# Autodesk Inventor assembly: montaje carro  extrusor
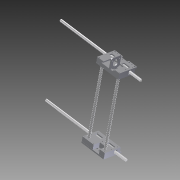
[picture p0: Inventor's stored thumbnail of the model, 180x180]
Saved by Autodesk Inventor 2012 (Build 160160000, 160)
## iProperties
Created: 2014-12-17
Part Number: montaje carro  extrusor
Document SubType Name: Assembly
Designer: PRINCIPAL
Author: PRINCIPAL
## Documents named in this file (16)
- \\LASERROUTERCNC\Users\Laser router cnc\Desktop\compartir con principal\impresora juan marc albert\montaje carro  extrusor.iam
- \\LASERROUTERCNC\Users\Laser router cnc\Desktop\compartir con principal\impresora juan marc albert\carro x lado polea pieza1.ipt
- \\LASERROUTERCNC\Users\Laser router cnc\Desktop\compartir con principal\impresora juan marc albert\carro x lado polea pieza2.ipt
- \\LASERROUTERCNC\Users\Laser router cnc\Desktop\compartir con principal\impresora juan marc albert\carro x lado polea pieza3.ipt
- \\LASERROUTERCNC\Users\Laser router cnc\Desktop\compartir con principal\impresora juan marc albert\carro x lado polea pieza4 tapa.ipt
- \\LASERROUTERCNC\Users\Laser router cnc\Desktop\compartir con principal\impresora juan marc albert\cojinete lm10uu.ipt
- \\LASERROUTERCNC\Users\Laser router cnc\Desktop\compartir con principal\impresora juan marc albert\carro x lado motor pieza 1.ipt
- \\LASERROUTERCNC\Users\Laser router cnc\Desktop\compartir con principal\impresora juan marc albert\carro x lado motor pieza 2 especial2.ipt
- \\LASERROUTERCNC\Users\Laser router cnc\Desktop\compartir con principal\impresora juan marc albert\carro x lado motor pieza 2parte 2.ipt
- \\LASERROUTERCNC\Users\Laser router cnc\Desktop\compartir con principal\impresora juan marc albert\carro x lado motor pieza 2parte 2-2.ipt
- \\LASERROUTERCNC\Users\Laser router cnc\Desktop\compartir con principal\impresora juan marc albert\carro x lado motor pieza 2parte 2-3.ipt
- \\LASERROUTERCNC\Users\Laser router cnc\Desktop\compartir con principal\impresora juan marc albert\carro x lado motor pieza 3.ipt
- \\LASERROUTERCNC\Users\Laser router cnc\Desktop\compartir con principal\impresora juan marc albert\carro x lado motor pieza 4.ipt
- \\LASERROUTERCNC\Users\Laser router cnc\Desktop\compartir con principal\impresora juan marc albert\carro x lado motor pieza 5 soporte nema.ipt
- \\LASERROUTERCNC\Users\Laser router cnc\Desktop\compartir con principal\impresora juan marc albert\varilla 10 carro x.ipt
- \\LASERROUTERCNC\Users\Laser router cnc\Desktop\compartir con principal\impresora juan marc albert\varilla 10 carro y.ipt
## Components (28 placed, 15 different names)
1. carro x lado polea pieza1:1 — Coincidencia:1, Coincidencia:2, Tangente:1, Tangente:2, Tangente:3, Tangente:4, Insertar:1, Insertar:2, Insertar:7, Insertar:8
2. carro x lado polea pieza2:1 — Insertar:7, Insertar:8, Insertar:9, Insertar:10, Insertar:45, Insertar:46
3. carro x lado polea pieza2:2 — Insertar:11, Insertar:12, Insertar:14
4. carro x lado polea pieza2:3 — Insertar:9, Insertar:10, Insertar:11, Insertar:12
5. carro x lado polea pieza3:1 — Insertar:5, Insertar:6, Insertar:13
6. carro x lado polea pieza3:2 — Insertar:3, Insertar:4, Insertar:5, Insertar:6
7. carro x lado polea pieza3:3 — Insertar:1, Insertar:2, Insertar:3, Insertar:4
8. carro x lado polea pieza4 tapa:1 — Insertar:13, Insertar:14
9. cojinete lm10uu:1 — Coincidencia:1, Tangente:3, Tangente:4
10. cojinete lm10uu:2 — Coincidencia:2, Tangente:1, Tangente:2, Insertar:48
11. carro x lado motor pieza 1:1 — Coincidencia:3, Coincidencia:4, Tangente:5, Tangente:6, Tangente:7, Tangente:8, Insertar:17, Insertar:18, Insertar:31, Insertar:32, Insertar:33, Insertar:34
12. carro x lado motor pieza 2 especial2:2 — Insertar:33, Insertar:34, Insertar:35, Insertar:36, Insertar:44
13. carro x lado motor pieza 2parte 2:1 — Insertar:29, Insertar:30, Insertar:41
14. carro x lado motor pieza 2parte 2:2 — Insertar:29, Insertar:30, Insertar:37, Insertar:38
15. carro x lado motor pieza 2parte 2-2:1 — Insertar:25, Insertar:26, Insertar:40
16. carro x lado motor pieza 2parte 2-2:2 — Insertar:25, Insertar:26, Insertar:35, Insertar:36
17. carro x lado motor pieza 2parte 2-3:1 — Insertar:31, Insertar:32, Insertar:37, Insertar:38, Insertar:42
18. carro x lado motor pieza 3:1 — Insertar:17, Insertar:18, Insertar:19, Insertar:20
19. carro x lado motor pieza 3:2 — Insertar:21, Insertar:22, Insertar:39
20. carro x lado motor pieza 3:3 — Insertar:19, Insertar:20, Insertar:21, Insertar:22
21. carro x lado motor pieza 4:1 — Insertar:39, Insertar:40, Insertar:41, Nivelación:1, Coincidencia:5, Coincidencia:6
22. carro x lado motor pieza 5 soporte nema:1 — Nivelación:1, Coincidencia:5, Coincidencia:6
23. cojinete lm10uu:3 — Coincidencia:4, Tangente:7, Tangente:8
24. cojinete lm10uu:4 — Coincidencia:3, Tangente:5, Tangente:6, Insertar:47
25. varilla 10 carro x:1 — Insertar:42, Insertar:46
26. varilla 10 carro x:2 — Insertar:44, Insertar:45
27. varilla 10 carro y:1 — Insertar:47
28. varilla 10 carro y:2 — Insertar:48
## Relationships (56: Insert 41, Tangent 8, Mate 6, Flush 1)
- Coincidencia:1 [Mate]: carro x lado polea pieza1:1 ↔ cojinete lm10uu:1
- Coincidencia:2 [Mate]: carro x lado polea pieza1:1 ↔ cojinete lm10uu:2
- Tangente:1: carro x lado polea pieza1:1 ↔ cojinete lm10uu:2
- Tangente:2: carro x lado polea pieza1:1 ↔ cojinete lm10uu:2
- Tangente:3: carro x lado polea pieza1:1 ↔ cojinete lm10uu:1
- Tangente:4: carro x lado polea pieza1:1 ↔ cojinete lm10uu:1
- Insertar:1: carro x lado polea pieza1:1 ↔ carro x lado polea pieza3:3
- Insertar:2: carro x lado polea pieza1:1 ↔ carro x lado polea pieza3:3
- Insertar:3: carro x lado polea pieza3:2 ↔ carro x lado polea pieza3:3
- Insertar:4: carro x lado polea pieza3:2 ↔ carro x lado polea pieza3:3
- Insertar:5: carro x lado polea pieza3:1 ↔ carro x lado polea pieza3:2
- Insertar:6: carro x lado polea pieza3:1 ↔ carro x lado polea pieza3:2
- Insertar:7: carro x lado polea pieza1:1 ↔ carro x lado polea pieza2:1
- Insertar:8: carro x lado polea pieza1:1 ↔ carro x lado polea pieza2:1
- Insertar:9: carro x lado polea pieza2:1 ↔ carro x lado polea pieza2:3
- Insertar:10: carro x lado polea pieza2:1 ↔ carro x lado polea pieza2:3
- Insertar:11: carro x lado polea pieza2:2 ↔ carro x lado polea pieza2:3
- Insertar:12: carro x lado polea pieza2:2 ↔ carro x lado polea pieza2:3
- Insertar:13: carro x lado polea pieza3:1 ↔ carro x lado polea pieza4 tapa:1
- Insertar:14: carro x lado polea pieza2:2 ↔ carro x lado polea pieza4 tapa:1
- Coincidencia:3 [Mate]: carro x lado motor pieza 1:1 ↔ cojinete lm10uu:4
- Coincidencia:4 [Mate]: carro x lado motor pieza 1:1 ↔ cojinete lm10uu:3
- Tangente:5: carro x lado motor pieza 1:1 ↔ cojinete lm10uu:4
- Tangente:6: carro x lado motor pieza 1:1 ↔ cojinete lm10uu:4
- Tangente:7: carro x lado motor pieza 1:1 ↔ cojinete lm10uu:3
- Tangente:8: carro x lado motor pieza 1:1 ↔ cojinete lm10uu:3
- Insertar:17: carro x lado motor pieza 1:1 ↔ carro x lado motor pieza 3:1
- Insertar:18: carro x lado motor pieza 1:1 ↔ carro x lado motor pieza 3:1
- Insertar:19: carro x lado motor pieza 3:1 ↔ carro x lado motor pieza 3:3
- Insertar:20: carro x lado motor pieza 3:1 ↔ carro x lado motor pieza 3:3
- Insertar:21: carro x lado motor pieza 3:2 ↔ carro x lado motor pieza 3:3
- Insertar:22: carro x lado motor pieza 3:2 ↔ carro x lado motor pieza 3:3
- Insertar:25: carro x lado motor pieza 2parte 2-2:1 ↔ carro x lado motor pieza 2parte 2-2:2
- Insertar:26: carro x lado motor pieza 2parte 2-2:1 ↔ carro x lado motor pieza 2parte 2-2:2
- Insertar:29: carro x lado motor pieza 2parte 2:1 ↔ carro x lado motor pieza 2parte 2:2
- Insertar:30: carro x lado motor pieza 2parte 2:1 ↔ carro x lado motor pieza 2parte 2:2
- Insertar:31: carro x lado motor pieza 1:1 ↔ carro x lado motor pieza 2parte 2-3:1
- Insertar:32: carro x lado motor pieza 1:1 ↔ carro x lado motor pieza 2parte 2-3:1
- Insertar:33: carro x lado motor pieza 1:1 ↔ carro x lado motor pieza 2 especial2:2
- Insertar:34: carro x lado motor pieza 1:1 ↔ carro x lado motor pieza 2 especial2:2
- Insertar:35: carro x lado motor pieza 2 especial2:2 ↔ carro x lado motor pieza 2parte 2-2:2
- Insertar:36: carro x lado motor pieza 2 especial2:2 ↔ carro x lado motor pieza 2parte 2-2:2
- Insertar:37: carro x lado motor pieza 2parte 2:2 ↔ carro x lado motor pieza 2parte 2-3:1
- Insertar:38: carro x lado motor pieza 2parte 2:2 ↔ carro x lado motor pieza 2parte 2-3:1
- Insertar:39: carro x lado motor pieza 3:2 ↔ carro x lado motor pieza 4:1
- Insertar:40: carro x lado motor pieza 2parte 2-2:1 ↔ carro x lado motor pieza 4:1
- Insertar:41: carro x lado motor pieza 2parte 2:1 ↔ carro x lado motor pieza 4:1
- Nivelación:1 [Flush]: carro x lado motor pieza 4:1 ↔ carro x lado motor pieza 5 soporte nema:1
- Coincidencia:5 [Mate]: carro x lado motor pieza 4:1 ↔ carro x lado motor pieza 5 soporte nema:1
- Insertar:42: carro x lado motor pieza 2parte 2-3:1 ↔ varilla 10 carro x:1
- Insertar:44: carro x lado motor pieza 2 especial2:2 ↔ varilla 10 carro x:2
- Insertar:45: carro x lado polea pieza2:1 ↔ varilla 10 carro x:2
- Insertar:46: carro x lado polea pieza2:1 ↔ varilla 10 carro x:1
- Coincidencia:6 [Mate]: carro x lado motor pieza 4:1 ↔ carro x lado motor pieza 5 soporte nema:1
- Insertar:47 (-65 mm): cojinete lm10uu:4 ↔ varilla 10 carro y:1
- Insertar:48 (-65 mm): cojinete lm10uu:2 ↔ varilla 10 carro y:2
